# Autodesk Inventor assembly: Cup_Dispenser
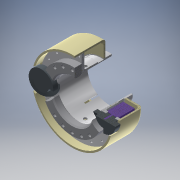
[picture p0: Inventor's stored thumbnail of the model, 180x180]
Saved by Autodesk Inventor 2016 (Build 200138000, 138)
## iProperties
Created: 2015-07-19
Part Number: Cup_Dispenser
Document SubType Name: Assembly
Designer: bastli
Author: bastli
## Documents named in this file (6)
- C:\Users\bastli\Documents\GitHub\BarBot\Conception\Mechanical\Cup_Dispenser_3\Cup_Dispenser.iam
- C:\Users\bastli\Documents\GitHub\BarBot\Conception\Mechanical\Cup_Dispenser_3\Fixture.ipt
- C:\Users\bastli\Documents\GitHub\BarBot\Conception\Mechanical\Cup_Dispenser_3\Transmission.ipt
- C:\Users\bastli\Documents\GitHub\BarBot\Conception\Mechanical\Cup_Dispenser_3\Nema 8.ipt
- C:\Users\bastli\Documents\GitHub\BarBot\Conception\Mechanical\Cup_Dispenser_3\Funnel_Adapter.ipt
- C:\Users\bastli\Documents\GitHub\BarBot\Conception\Mechanical\Cup_Dispenser_3\Hull.ipt
## Components (8 placed, 5 different names)
1. Fixture:1 — Rigid:1, Rigid:3, Flush:1, Rotational:3, Flush:2
2. Transmission:1 — Rotational:1
3. Nema 8:1 — Rigid:1, Rotational:1
4. Nema 8:2 — Rigid:3, Rotational:2
5. Transmission:2 — Rotational:2
6. Funnel_Adapter:1 — Flush:1
7. Funnel_Adapter:2 — Rotational:3
8. Hull:1 — Flush:2
## Relationships (7: RevoluteJoint 3, WeldJoint 2, Flush 2)
- Rigid:1 [WeldJoint]: Fixture:1 ↔ Nema 8:1
- Rotational:1 [RevoluteJoint]: Transmission:1 ↔ Nema 8:1
- Rigid:3 [WeldJoint]: Fixture:1 ↔ Nema 8:2
- Rotational:2 [RevoluteJoint]: Nema 8:2 ↔ Transmission:2
- Flush:1: Fixture:1 ↔ Funnel_Adapter:1
- Rotational:3 [RevoluteJoint]: Fixture:1 ↔ Funnel_Adapter:2
- Flush:2: Fixture:1 ↔ Hull:1
